# Autodesk Inventor assembly: PartsAssembly
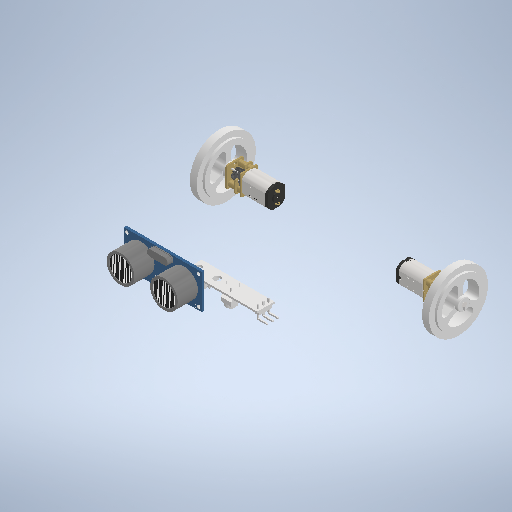
[picture p0: Inventor's stored thumbnail of the model, 512x512]
Saved by Autodesk Inventor 2025.1 (Build 291241020, 241B)
## iProperties
Created: 2024-12-27
Part Number: PartsAssembly
Document SubType Name: Assembly
Designer: herme
Author: herme
## Documents named in this file (5)
- C:\Users\herme\Documents\Sumobot\CAD\PartsAssembly.iam
- C:\Users\herme\Documents\Sumobot\CAD\Kit Parts\Motor.iam
- C:\Users\herme\Documents\Sumobot\CAD\Kit Parts\Wheel 34mm.ipt
- C:\Users\herme\Documents\Sumobot\CAD\Kit Parts\IRSensor.ipt
- C:\Users\herme\Documents\Sumobot\CAD\Kit Parts\UltrasonicSensor.iam
## Components (6 placed, 4 different names)
1. Wheel 34mm:1 — Insert:2
2. Wheel 34mm:2 — Insert:1
3. Motor:1 [sub-assembly] — Insert:1
4. Motor:2 [sub-assembly] — Insert:2
5. IRSensor:2
6. UltrasonicSensor:1 [sub-assembly]
## Relationships (2: Insert 2)
- Insert:1: Wheel 34mm:2 ↔ Motor:1
- Insert:2: Wheel 34mm:1 ↔ Motor:2
